# Autodesk Inventor assembly: solids feeder assembly
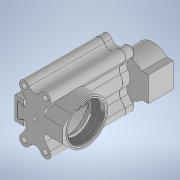
[picture p0: Inventor's stored thumbnail of the model, 180x180]
Saved by Autodesk Inventor 2022 (Build 260153000, 153)
## iProperties
Created: 2022-11-12
Part Number: solids feeder assembly
Document SubType Name: Assembly
Designer: efred
Author: efred
## Documents named in this file (8)
- C:\Users\efred\OneDrive - Imperial College London\ROBOICP MK2\solids feeder assembly.iam
- C:\Users\efred\OneDrive - Imperial College London\ROBOICP MK2\Screw Shaft.ipt
- C:\Users\efred\OneDrive - Imperial College London\ROBOICP MK2\smol stepper.ipt
- C:\Users\efred\OneDrive - Imperial College London\ROBOICP MK2\screw_casing.ipt
- C:\Users\efred\OneDrive - Imperial College London\ROBOICP MK2\shaft encap lid.ipt
- C:\Users\efred\OneDrive - Imperial College London\ROBOICP MK2\vial thread insert.ipt
- C:\Users\efred\OneDrive - Imperial College London\ROBOICP MK2\spout.ipt
- C:\Users\efred\OneDrive - Imperial College London\ROBOICP MK2\dovetail insert.ipt
## Components (7 placed, 7 different names)
1. Screw Shaft:1 — Mate:4, Flush:10, Mate:7, Mate:10
2. smol stepper:1 — Mate:4, Mate:10, Flush:12, Flush:13
3. screw_casing:1 — Flush:2, Flush:3, Flush:11, Mate:7, Mate:8, Mate:9, Flush:14, Flush:17
4. shaft encap lid:1 — Flush:4, Flush:12, Flush:13
5. vial thread insert:1 — Mate:8, Mate:9
6. spout:1 — Flush:15, Flush:16
7. dovetail insert:1 — Flush:17
## Relationships (16: Flush 11, Mate 5)
- Mate:4: Screw Shaft:1 ↔ smol stepper:1
- Flush:2: screw_casing:1
- Flush:3 (0.1 mm): screw_casing:1
- Flush:4: shaft encap lid:1
- Flush:10 (0.1 mm): Screw Shaft:1
- Flush:11 (0.1 mm): screw_casing:1
- Mate:7 (0.2 mm): Screw Shaft:1 ↔ screw_casing:1
- Mate:8 (0.1 mm): screw_casing:1 ↔ vial thread insert:1
- Mate:9: screw_casing:1 ↔ vial thread insert:1
- Mate:10 (0.1 mm): Screw Shaft:1 ↔ smol stepper:1
- Flush:12 (0.1 mm): smol stepper:1 ↔ shaft encap lid:1
- Flush:13 (0.1 mm): smol stepper:1 ↔ shaft encap lid:1
- Flush:14 (0.1 mm): screw_casing:1
- Flush:15: spout:1
- Flush:16: spout:1
- Flush:17: screw_casing:1 ↔ dovetail insert:1
